# Autodesk Inventor assembly: 141
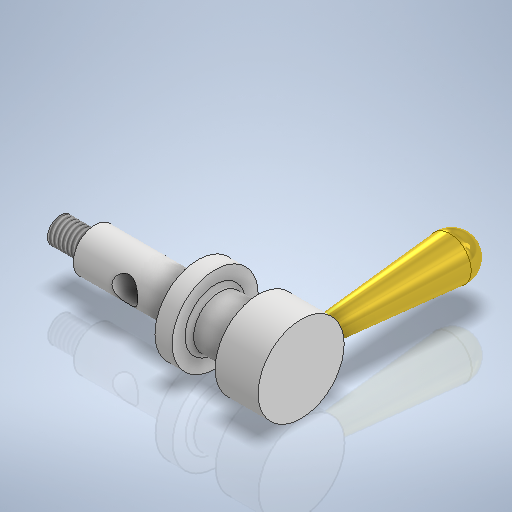
[picture p0: Inventor's stored thumbnail of the model, 512x512]
Saved by Autodesk Inventor 2025.1 (Build 291241000, 241)
## iProperties
Created: 2024-08-05
Part Number: 141
Document SubType Name: Assembly
Designer: ffogue
Author: ffogue
## Documents named in this file (3)
- C:\Projkete - Übungen\Freedom\141.iam
- C:\Projkete - Übungen\Freedom\141.ipt
- C:\Projkete - Übungen\Freedom\134 handle.ipt
## Components (2 placed, 2 different names)
1. 141:1 — Mate:1, Insert:1
2. 134 handle:1 — Mate:1, Insert:1
## Relationships (2: Mate 1, Insert 1)
- Mate:1: 141:1 ↔ 134 handle:1
- Insert:1: 141:1 ↔ 134 handle:1
